# Autodesk Inventor assembly: Roller-ver21-1111-2021
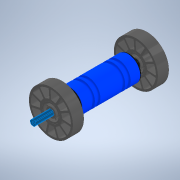
[picture p0: Inventor's stored thumbnail of the model, 180x180]
Saved by Autodesk Inventor 2020 (Build 240168000, 168)
## iProperties
Created: 2021-01-26
Part Number: Roller-ver21-1111-2021
Document SubType Name: Assembly
Designer: Caitlin
Author: Caitlin
## Documents named in this file (6)
- D:\PHRC CADD 2021\PHRC CADD\2020 Infinite Recharge\2021 Infinite Recharge\Chassis\Roller-ver21-1111-2021.iam
- D:\PHRC CADD 2021\PHRC CADD\2020 Infinite Recharge\Storage\Parts\Roller-ver3-1111-2019.ipt
- D:\PHRC CADD 2021\PHRC CADD\Resources\VEXpro Resources\Versa Motion\VersaHub(0.5inHex)-1111-2016.ipt
- D:\PHRC CADD 2021\PHRC CADD\Resources\VEXpro Resources\Wheels\4 inch\4IN-CompliantWheel-500Hex.iam
- D:\PHRC CADD 2021\PHRC CADD\2020 Infinite Recharge\2021 Infinite Recharge\Chassis\0.5inThunderHexShaft(12in))-1111-2021.ipt
- D:\PHRC CADD 2021\PHRC CADD\Resources\VEXpro Resources\Spacers\0.25inAcetalSpacer(0.5inHex)-1111-2016.ipt
## Components (8 placed, 5 different names)
1. 0.5inThunderHexShaft(12in))-1111-2021:1 — Cylindrical:5, Flush:2, Angle:3, Angle:4, Cylindrical:6, Angle:5, Cylindrical:7, Angle:6, Cylindrical:8, Angle:7, Cylindrical:9, Angle:8
2. Roller-ver3-1111-2019:2 — Cylindrical:5, Flush:2, Rotational:1, Rotational:2
3. VersaHub(0.5inHex)-1111-2016:3 — Rotational:1, Angle:3, Mate:2
4. VersaHub(0.5inHex)-1111-2016:4 — Rotational:2, Angle:4, Mate:1
5. 0.25inAcetalSpacer(0.5inHex)-1111-2016:1 — Cylindrical:6, Angle:5, Mate:1, Mate:4
6. 0.25inAcetalSpacer(0.5inHex)-1111-2016:2 — Cylindrical:7, Angle:6, Mate:2, Mate:3
7. 4IN-CompliantWheel-500Hex:1 [sub-assembly] — Cylindrical:8, Angle:7, Mate:3
8. 4IN-CompliantWheel-500Hex:2 [sub-assembly] — Cylindrical:9, Angle:8, Mate:4
## Relationships (18: Angle 6, CylindricalJoint 5, Mate 4, RevoluteJoint 2, Flush 1)
- Cylindrical:5: 0.5inThunderHexShaft(12in))-1111-2021:1 ↔ Roller-ver3-1111-2019:2
- Flush:2 (85.725 mm): 0.5inThunderHexShaft(12in))-1111-2021:1 ↔ Roller-ver3-1111-2019:2
- Rotational:1 [RevoluteJoint]: Roller-ver3-1111-2019:2 ↔ VersaHub(0.5inHex)-1111-2016:3
- Angle:3 (0 deg): 0.5inThunderHexShaft(12in))-1111-2021:1 ↔ VersaHub(0.5inHex)-1111-2016:3
- Rotational:2 [RevoluteJoint]: Roller-ver3-1111-2019:2 ↔ VersaHub(0.5inHex)-1111-2016:4
- Angle:4 (0 deg): 0.5inThunderHexShaft(12in))-1111-2021:1 ↔ VersaHub(0.5inHex)-1111-2016:4
- Cylindrical:6: 0.5inThunderHexShaft(12in))-1111-2021:1 ↔ 0.25inAcetalSpacer(0.5inHex)-1111-2016:1
- Angle:5 (90 deg): 0.5inThunderHexShaft(12in))-1111-2021:1 ↔ 0.25inAcetalSpacer(0.5inHex)-1111-2016:1
- Mate:1: VersaHub(0.5inHex)-1111-2016:4 ↔ 0.25inAcetalSpacer(0.5inHex)-1111-2016:1
- Cylindrical:7: 0.5inThunderHexShaft(12in))-1111-2021:1 ↔ 0.25inAcetalSpacer(0.5inHex)-1111-2016:2
- Angle:6 (90 deg): 0.5inThunderHexShaft(12in))-1111-2021:1 ↔ 0.25inAcetalSpacer(0.5inHex)-1111-2016:2
- Mate:2: VersaHub(0.5inHex)-1111-2016:3 ↔ 0.25inAcetalSpacer(0.5inHex)-1111-2016:2
- Cylindrical:8: 0.5inThunderHexShaft(12in))-1111-2021:1 ↔ 4IN-CompliantWheel-500Hex:1
- Angle:7 (90 deg): 0.5inThunderHexShaft(12in))-1111-2021:1 ↔ 4IN-CompliantWheel-500Hex:1
- Mate:3: 0.25inAcetalSpacer(0.5inHex)-1111-2016:2 ↔ 4IN-CompliantWheel-500Hex:1
- Cylindrical:9: 0.5inThunderHexShaft(12in))-1111-2021:1 ↔ 4IN-CompliantWheel-500Hex:2
- Angle:8 (90 deg): 0.5inThunderHexShaft(12in))-1111-2021:1 ↔ 4IN-CompliantWheel-500Hex:2
- Mate:4: 0.25inAcetalSpacer(0.5inHex)-1111-2016:1 ↔ 4IN-CompliantWheel-500Hex:2
